# Autodesk Inventor assembly: ElevatorClaw
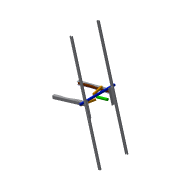
[picture p0: Inventor's stored thumbnail of the model, 180x180]
Saved by Autodesk Inventor 2015 (Build 190159000, 159)
## iProperties
Created: 2015-01-10
Part Number: ElevatorClaw
Document SubType Name: Assembly
Designer: Tanner
Author: Tanner
## Documents named in this file (5)
- C:\Users\Tanner\Documents\Inventor\ElevatorCar\ElevatorClaw.iam
- C:\Users\Tanner\Documents\Inventor\ElevatorCAD\Kevin'sCustomUnistrut.ipt
- C:\Users\Tanner\Documents\Claw\ClawV2assm.iam
- C:\Users\Tanner\Documents\Inventor\ElevatorCAD\Elevatorcarv2.iam
- C:\Users\Tanner\Documents\Inventor\ElevatorCAD\CarLbraket.ipt
## Components (7 placed, 4 different names)
1. Kevin'sCustomUnistrut:2 — Flush:17, Flush:22, Tangent:4, Tangent:5, Tangent:6, Flush:27, Flush:28, Flush:29
2. Kevin'sCustomUnistrut:3 — Flush:17, Flush:22, Flush:27, Flush:28, Tangent:7
3. ClawV2assm:1 [sub-assembly] — Mate:5, Flush:29, Flush:30, Mate:6, Flush:31
4. Elevatorcarv2:1 [sub-assembly] — Flush:32, Mate:7, Flush:33, Tangent:7
5. Elevatorcarv2:3 [sub-assembly] — Tangent:4, Tangent:5, Tangent:6, Mate:2, Flush:25, Flush:26
6. CarLbraket:1 — Mate:2, Flush:25, Flush:26, Mate:4, Mate:5, Flush:30
7. CarLbraket:2 — Mate:4, Mate:6, Flush:31, Flush:32, Mate:7, Flush:33
## Relationships (20: Flush 11, Mate 5, Tangent 4)
- Flush:17: Kevin'sCustomUnistrut:2 ↔ Kevin'sCustomUnistrut:3
- Flush:22: Kevin'sCustomUnistrut:2 ↔ Kevin'sCustomUnistrut:3
- Tangent:4: Kevin'sCustomUnistrut:2 ↔ Elevatorcarv2:3
- Tangent:5: Kevin'sCustomUnistrut:2 ↔ Elevatorcarv2:3
- Tangent:6: Kevin'sCustomUnistrut:2 ↔ Elevatorcarv2:3
- Mate:2: Elevatorcarv2:3 ↔ CarLbraket:1
- Flush:25: Elevatorcarv2:3 ↔ CarLbraket:1
- Flush:26: Elevatorcarv2:3 ↔ CarLbraket:1
- Flush:27: Kevin'sCustomUnistrut:2 ↔ Kevin'sCustomUnistrut:3
- Flush:28: Kevin'sCustomUnistrut:2 ↔ Kevin'sCustomUnistrut:3
- Mate:4 (432.7144 mm): CarLbraket:1 ↔ CarLbraket:2
- Mate:5: ClawV2assm:1 ↔ CarLbraket:1
- Flush:29 (60.198 mm): Kevin'sCustomUnistrut:2 ↔ ClawV2assm:1
- Flush:30: ClawV2assm:1 ↔ CarLbraket:1
- Mate:6: ClawV2assm:1 ↔ CarLbraket:2
- Flush:31: ClawV2assm:1 ↔ CarLbraket:2
- Flush:32: Elevatorcarv2:1 ↔ CarLbraket:2
- Mate:7: Elevatorcarv2:1 ↔ CarLbraket:2
- Flush:33: Elevatorcarv2:1 ↔ CarLbraket:2
- Tangent:7: Kevin'sCustomUnistrut:3 ↔ Elevatorcarv2:1
